# Autodesk Inventor assembly: ftc robot
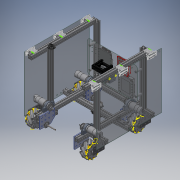
[picture p0: Inventor's stored thumbnail of the model, 180x180]
Saved by Autodesk Inventor 2017 (Build 210142000, 142)
## iProperties
Created: 2017-06-13
Part Number: ftc robot
Document SubType Name: Assembly
Designer: slong
Author: slong
## Documents named in this file (25)
- C:\Users\sfreisem-kirov\Documents\GitHub\ftc_app\Parts\ftc robot\ftc robot.iam
- C:\Users\sfreisem-kirov\Documents\GitHub\ftc_app\Parts\ftc robot\10HoleExtrudedPlate.STL.ipt
- C:\Users\sfreisem-kirov\Documents\GitHub\ftc_app\Parts\ftc robot\100mm Aluminum Mecanum wheels.ipt
- C:\Users\sfreisem-kirov\Documents\GitHub\ftc_app\Parts\ftc robot\extruded aluminum (4in).ipt
- C:\Users\sfreisem-kirov\Documents\GitHub\ftc_app\Parts\ftc robot\extruded aluminum (vertical).ipt
- C:\Users\sfreisem-kirov\Documents\GitHub\ftc_app\Parts\ftc robot\extruded aluminum (horizontal).ipt
- C:\Users\sfreisem-kirov\Documents\GitHub\ftc_app\Parts\ftc robot\8020 L bracket.ipt
- C:\Users\sfreisem-kirov\Documents\GitHub\ftc_app\Parts\ftc robot\Motor Bracket.ipt
- C:\Users\sfreisem-kirov\Documents\GitHub\ftc_app\Parts\ftc robot\Andymark Motor.ipt
- C:\Users\sfreisem-kirov\Documents\GitHub\ftc_app\Parts\ftc robot\8020 small L bracket.ipt
- C:\Users\sfreisem-kirov\Documents\GitHub\ftc_app\Parts\ftc robot\extracted\tetrix_739079_2012.iam
- C:\Users\sfreisem-kirov\Documents\GitHub\ftc_app\Parts\ftc robot\175mm 6mm D axle.ipt
- C:\Users\sfreisem-kirov\Documents\GitHub\ftc_app\Parts\ftc robot\extracted\tetrix_739165_2012.ipt
- C:\Users\sfreisem-kirov\Documents\GitHub\ftc_app\Parts\ftc robot\circuit board correct.ipt
- C:\Users\sfreisem-kirov\Documents\GitHub\ftc_app\Parts\ftc robot\MRI45-2200_Power_Distribution_Module.ipt
- C:\Users\sfreisem-kirov\Documents\GitHub\ftc_app\Parts\ftc robot\MRI45-2203_Motor_Controller.ipt
- C:\Users\sfreisem-kirov\Documents\GitHub\ftc_app\Parts\ftc robot\MRI45-2204_Servo_Controller.ipt
- C:\Users\sfreisem-kirov\Documents\GitHub\ftc_app\Parts\ftc robot\spacer2.ipt
- C:\Users\sfreisem-kirov\Documents\GitHub\ftc_app\Parts\ftc robot\45-2003_Compass.ipt
- C:\Users\sfreisem-kirov\Documents\GitHub\ftc_app\Parts\ftc robot\45-2018_Color.ipt
- C:\Users\sfreisem-kirov\Documents\GitHub\ftc_app\Parts\ftc robot\extracted\tetrix_739070_2012.ipt
- C:\Users\sfreisem-kirov\Documents\GitHub\ftc_app\Parts\ftc robot\side shield.ipt
- C:\Users\sfreisem-kirov\Documents\GitHub\ftc_app\Parts\ftc robot\45-2017_IRSeekerV3.ipt
- C:\Users\sfreisem-kirov\Documents\GitHub\ftc_app\Parts\ftc robot\ShieldSlideAttachment2-SFK.ipt
- C:\Users\sfreisem-kirov\Documents\GitHub\ftc_app\Parts\phoneHolder\PhoneFlipper1-SFK.iam
## Components (81 placed, 24 different names)
1. 10HoleExtrudedPlate.STL:1 — Mate:7, Mate:8, Flush:10, Mate:33, Mate:65
2. 10HoleExtrudedPlate.STL:2 — Mate:9, Mate:10, Flush:10, Flush:16, Mate:20, Mate:70
3. 10HoleExtrudedPlate.STL:3 — Mate:14, Flush:15, Mate:16, Flush:18, Mate:56, Mate:64
4. 10HoleExtrudedPlate.STL:4 — Mate:13, Flush:14, Flush:16, Flush:18, Mate:18, Mate:19, Mate:68
5. 100mm Aluminum Mecanum wheels:1 — Mate:20, Mate:29, Mate:30, Rotation:7
6. 100mm Aluminum Mecanum wheels:2 — Mate:22, Mate:25, Mate:26, Rotation:2
7. 100mm Aluminum Mecanum wheels:3 — Mate:19, Mate:27, Mate:28, Rotation:8
8. 100mm Aluminum Mecanum wheels:4 — Mate:23, Mate:24, Rotation:6
9. extruded aluminum (4in):1 — Flush:11, Mate:11, Flush:13, Mate:17, Flush:19, Mate:50, Flush:35, Flush:66
10. extruded aluminum (4in):2 — Mate:12, Flush:12, Flush:13, Mate:15, Flush:17, Mate:48, Flush:34
11. extruded aluminum (vertical):1 — Mate:50, Mate:51, Flush:35
12. extruded aluminum (vertical):2 — Mate:48, Mate:49, Flush:34, Mate:122, Flush:69, Flush:70
13. extruded aluminum (vertical):3 — Mate:46, Flush:33, Mate:97, Mate:112
14. extruded aluminum (vertical):4 — Mate:44, Mate:45, Flush:32, Flush:46, Mate:98, Mate:111
15. extruded aluminum (horizontal):1 — Mate:2, Flush:2, Flush:3, Mate:3, Mate:8, Mate:12, Flush:12, Mate:14, Flush:15, Mate:36, Mate:37, Flush:23, Flush:24, Mate:44, Mate:49, Mate:53, Flush:58, Mate:119
16. extruded aluminum (horizontal):2 — Mate:1, Flush:1, Mate:2, Flush:2, Flush:4, Flush:5, Mate:4, Flush:6, Flush:7, Mate:5, Flush:8, Flush:9, Mate:45, Flush:32, Mate:46, Mate:113
17. extruded aluminum (horizontal):3 — Mate:1, Flush:1, Flush:3, Flush:4, Mate:9, Flush:11, Mate:11, Mate:13, Flush:14, Flush:22, Mate:34, Mate:35, Flush:25, Flush:33, Mate:51, Mate:54, Mate:97, Flush:57, Mate:117
18. extruded aluminum (horizontal):4 — Mate:3, Flush:5, Mate:52, Flush:36, Flush:37, Mate:55, Mate:113, Mate:114, Flush:59, Flush:62, Mate:118, Flush:63, Mate:120, Mate:121
19. 8020 L bracket:1 — Mate:5, Flush:8, Flush:9, Mate:10, Flush:30, Mate:58, Flush:41
20. 8020 L bracket:2 — Mate:15, Flush:17, Mate:16, Mate:22, Mate:31, Flush:29, Flush:38
21. 8020 L bracket:3 — Mate:4, Flush:6, Flush:7, Mate:7, Flush:28, Mate:59, Flush:39
22. 8020 L bracket:4 — Mate:17, Flush:19, Mate:18, Mate:32, Flush:31, Mate:57, Flush:40
23. Motor Bracket:1 — Mate:36, Flush:24, Flush:26, Mate:40
24. Motor Bracket:2 — Mate:37, Flush:23, Flush:27, Mate:41
25. Motor Bracket:3 — Mate:35, Flush:25, Flush:26, Mate:39
26. Motor Bracket:4 — Flush:22, Mate:34, Flush:27, Mate:38
27. Andymark Motor:1 — Mate:38, Mate:43, Flush:30, Mate:72, Mate:94
28. Andymark Motor:2 — Mate:39, Mate:42, Flush:31, Mate:69, Mate:76
29. Andymark Motor:3 — Mate:40, Mate:42, Flush:29, Mate:63, Mate:82
30. Andymark Motor:4 — Mate:41, Mate:43, Flush:28, Mate:67, Mate:88
31. 8020 small L bracket:1 — Mate:54, Flush:37, Mate:55
32. 8020 small L bracket:4 — Mate:52, Flush:36, Mate:53
33. tetrix_739079_2012:1 [sub-assembly] — Mate:25, Mate:26, Flush:21, Mate:31
34. tetrix_739079_2012:2 [sub-assembly] — Mate:23, Mate:24, Flush:21, Mate:33
35. tetrix_739079_2012:3 [sub-assembly] — Mate:27, Mate:28, Flush:20, Mate:32
36. tetrix_739079_2012:4 [sub-assembly] — Mate:29, Mate:30, Flush:20
37. tetrix_739079_2012:5 [sub-assembly] — Mate:60, Flush:42, Rotation:1, Rotation:2, Mate:64, Mate:80, Mate:81
38. tetrix_739079_2012:6 [sub-assembly] — Mate:69, Flush:44, Rotation:4, Mate:77, Mate:78
39. tetrix_739079_2012:7 [sub-assembly] — Mate:61, Mate:68, Flush:44, Rotation:4, Rotation:8, Mate:73, Mate:74, Mate:75
40. tetrix_739079_2012:9 [sub-assembly] — Mate:65, Mate:66, Flush:43, Rotation:5, Rotation:6, Mate:86, Mate:87
41. tetrix_739079_2012:10 [sub-assembly] — Mate:67, Flush:43, Rotation:5, Mate:89, Mate:90
42. tetrix_739079_2012:11 [sub-assembly] — Mate:70, Mate:71, Flush:45, Rotation:3, Rotation:7, Mate:92, Mate:93
43. tetrix_739079_2012:12 [sub-assembly] — Mate:72, Flush:45, Rotation:3, Mate:95, Mate:96
44. tetrix_739079_2012:8 [sub-assembly] — Mate:63, Flush:42, Rotation:1, Mate:83, Mate:84
45. 175mm 6mm D axle:1 — Mate:56, Flush:38, Mate:60, Mate:79
46. 175mm 6mm D axle:2 — Mate:57, Flush:40, Mate:61
47. 175mm 6mm D axle:3 — Mate:59, Flush:39, Mate:66, Mate:85
48. 175mm 6mm D axle:4 — Mate:58, Flush:41, Mate:71, Mate:91
49. tetrix_739165_2012:1 — Mate:76, Mate:77, Mate:78
50. tetrix_739165_2012:2 — Mate:85, Mate:86, Mate:87
51. tetrix_739165_2012:3 — Mate:91, Mate:92, Mate:93
52. tetrix_739165_2012:4 — Mate:82, Mate:83, Mate:84
53. tetrix_739165_2012:5 — Mate:79, Mate:80, Mate:81
54. tetrix_739165_2012:6 — Mate:88, Mate:89, Mate:90
55. tetrix_739165_2012:7 — Mate:94, Mate:95, Mate:96
56. tetrix_739165_2012:8 — Mate:73, Mate:74, Mate:75
57. circuit board correct:1 — Flush:46, Mate:98, Mate:99, Flush:47, Flush:48, Mate:100, Mate:101, Mate:102, Flush:49, Flush:50, Flush:51, Flush:52, Flush:53, Flush:54, Mate:103, Mate:104, Mate:105, Mate:106, Mate:107, Mate:108, Mate:109, Mate:110
58. MRI45-2200_Power_Distribution_Module:1 — Mate:99, Flush:47, Flush:48
59. MRI45-2203_Motor_Controller:1 — Mate:100, Flush:49, Flush:50
60. MRI45-2203_Motor_Controller:2 — Mate:101, Flush:53, Flush:54
61. MRI45-2204_Servo_Controller:1 — Mate:102, Flush:51, Flush:52
62. spacer2:1 — Mate:106, Mate:108
63. spacer2:2 — Mate:105, Mate:107
64. spacer2:3 — Mate:103, Mate:109
65. spacer2:4 — Mate:104, Mate:110
66. extruded aluminum (horizontal):7 — Mate:111, Flush:55, Flush:58, Flush:67, Flush:68, Mate:132, Mate:133, Mate:134
67. extruded aluminum (horizontal):8 — Mate:112, Flush:55, Flush:57, Flush:65, Mate:126, Mate:135, Mate:136, Mate:137, Mate:138
68. 45-2003_Compass:1 — Mate:117, Mate:118, Flush:63
69. 45-2018_Color:1 — Mate:115, Flush:60, Flush:61, Mate:116, Mate:119
70. 45-2018_Color:2 — Mate:115, Flush:60, Flush:61, Flush:62
71. tetrix_739070_2012:1 — Mate:114, Flush:59, Mate:116
72. side shield:2 — Mate:120, Flush:65, Flush:66, Mate:125, Mate:127, Mate:128
73. side shield:3 — Mate:121, Flush:67, Flush:68, Mate:129, Mate:130, Mate:131
74. 45-2017_IRSeekerV3:1 — Mate:122, Flush:69, Flush:70
75. ShieldSlideAttachment2-SFK:1 — Mate:125, Mate:126
76. ShieldSlideAttachment2-SFK:2 — Mate:128, Mate:136
77. ShieldSlideAttachment2-SFK:3 — Mate:129, Mate:132
78. ShieldSlideAttachment2-SFK:4 — Mate:127, Mate:135
79. ShieldSlideAttachment2-SFK:5 — Mate:131, Mate:133
80. ShieldSlideAttachment2-SFK:6 — Mate:130, Mate:134
81. PhoneFlipper1-SFK:1 [sub-assembly] — Mate:137, Mate:138
## Relationships (208: Mate 132, Flush 68, RelateRotation 8)
- Mate:1: extruded aluminum (horizontal):2 ↔ extruded aluminum (horizontal):3
- Flush:1 (-76.2 mm): extruded aluminum (horizontal):2 ↔ extruded aluminum (horizontal):3
- Mate:2: extruded aluminum (horizontal):1 ↔ extruded aluminum (horizontal):2
- Flush:2 (-76.2 mm): extruded aluminum (horizontal):1 ↔ extruded aluminum (horizontal):2
- Flush:3: extruded aluminum (horizontal):1 ↔ extruded aluminum (horizontal):3
- Flush:4: extruded aluminum (horizontal):2 ↔ extruded aluminum (horizontal):3
- Mate:3: extruded aluminum (horizontal):1 ↔ extruded aluminum (horizontal):4
- Flush:5: extruded aluminum (horizontal):2 ↔ extruded aluminum (horizontal):4
- Mate:4: extruded aluminum (horizontal):2 ↔ 8020 L bracket:3
- Flush:6: extruded aluminum (horizontal):2 ↔ 8020 L bracket:3
- Flush:7: extruded aluminum (horizontal):2 ↔ 8020 L bracket:3
- Mate:5: extruded aluminum (horizontal):2 ↔ 8020 L bracket:1
- Flush:8: extruded aluminum (horizontal):2 ↔ 8020 L bracket:1
- Flush:9: extruded aluminum (horizontal):2 ↔ 8020 L bracket:1
- Mate:7: 10HoleExtrudedPlate.STL:1 ↔ 8020 L bracket:3
- Mate:8: 10HoleExtrudedPlate.STL:1 ↔ extruded aluminum (horizontal):1
- Mate:9: 10HoleExtrudedPlate.STL:2 ↔ extruded aluminum (horizontal):3
- Mate:10: 10HoleExtrudedPlate.STL:2 ↔ 8020 L bracket:1
- Flush:10: 10HoleExtrudedPlate.STL:1 ↔ 10HoleExtrudedPlate.STL:2
- Flush:11: extruded aluminum (4in):1 ↔ extruded aluminum (horizontal):3
- Mate:11: extruded aluminum (4in):1 ↔ extruded aluminum (horizontal):3
- Mate:12: extruded aluminum (4in):2 ↔ extruded aluminum (horizontal):1
- Flush:12: extruded aluminum (4in):2 ↔ extruded aluminum (horizontal):1
- Flush:13: extruded aluminum (4in):1 ↔ extruded aluminum (4in):2
- Mate:13: 10HoleExtrudedPlate.STL:4 ↔ extruded aluminum (horizontal):3
- Flush:14: 10HoleExtrudedPlate.STL:4 ↔ extruded aluminum (horizontal):3
- Mate:14: 10HoleExtrudedPlate.STL:3 ↔ extruded aluminum (horizontal):1
- Flush:15: 10HoleExtrudedPlate.STL:3 ↔ extruded aluminum (horizontal):1
- Flush:16: 10HoleExtrudedPlate.STL:2 ↔ 10HoleExtrudedPlate.STL:4
- Mate:15: extruded aluminum (4in):2 ↔ 8020 L bracket:2
- Flush:17: extruded aluminum (4in):2 ↔ 8020 L bracket:2
- Mate:16: 10HoleExtrudedPlate.STL:3 ↔ 8020 L bracket:2
- Flush:18: 10HoleExtrudedPlate.STL:3 ↔ 10HoleExtrudedPlate.STL:4
- Mate:17: extruded aluminum (4in):1 ↔ 8020 L bracket:4
- Flush:19: extruded aluminum (4in):1 ↔ 8020 L bracket:4
- Mate:18: 10HoleExtrudedPlate.STL:4 ↔ 8020 L bracket:4
- Mate:19: 10HoleExtrudedPlate.STL:4 ↔ 100mm Aluminum Mecanum wheels:3
- Mate:20: 10HoleExtrudedPlate.STL:2 ↔ 100mm Aluminum Mecanum wheels:1
- Mate:22: 100mm Aluminum Mecanum wheels:2 ↔ 8020 L bracket:2
- Mate:23: 100mm Aluminum Mecanum wheels:4 ↔ tetrix_739079_2012:2
- Mate:24: 100mm Aluminum Mecanum wheels:4 ↔ tetrix_739079_2012:2
- Mate:25: 100mm Aluminum Mecanum wheels:2 ↔ tetrix_739079_2012:1
- Mate:26: 100mm Aluminum Mecanum wheels:2 ↔ tetrix_739079_2012:1
- Mate:27: 100mm Aluminum Mecanum wheels:3 ↔ tetrix_739079_2012:3
- Mate:28: 100mm Aluminum Mecanum wheels:3 ↔ tetrix_739079_2012:3
- Mate:29: 100mm Aluminum Mecanum wheels:1 ↔ tetrix_739079_2012:4
- Mate:30: 100mm Aluminum Mecanum wheels:1 ↔ tetrix_739079_2012:4
- Flush:20: tetrix_739079_2012:3 ↔ tetrix_739079_2012:4
- Flush:21: tetrix_739079_2012:1 ↔ tetrix_739079_2012:2
- Mate:31: 8020 L bracket:2 ↔ tetrix_739079_2012:1
- Mate:32: 8020 L bracket:4 ↔ tetrix_739079_2012:3
- Mate:33: 10HoleExtrudedPlate.STL:1 ↔ tetrix_739079_2012:2
- Flush:22 (6.35 mm): extruded aluminum (horizontal):3 ↔ Motor Bracket:4
- Mate:34: extruded aluminum (horizontal):3 ↔ Motor Bracket:4
- Mate:35: extruded aluminum (horizontal):3 ↔ Motor Bracket:3
- Mate:36: extruded aluminum (horizontal):1 ↔ Motor Bracket:1
- Mate:37: extruded aluminum (horizontal):1 ↔ Motor Bracket:2
- Flush:23 (6.35 mm): extruded aluminum (horizontal):1 ↔ Motor Bracket:2
- Flush:24 (6.35 mm): extruded aluminum (horizontal):1 ↔ Motor Bracket:1
- Flush:25 (6.35 mm): extruded aluminum (horizontal):3 ↔ Motor Bracket:3
- Flush:26: Motor Bracket:1 ↔ Motor Bracket:3
- Flush:27: Motor Bracket:2 ↔ Motor Bracket:4
- Mate:38: Motor Bracket:4 ↔ Andymark Motor:1
- Mate:39: Motor Bracket:3 ↔ Andymark Motor:2
- Mate:40: Motor Bracket:1 ↔ Andymark Motor:3
- Mate:41: Motor Bracket:2 ↔ Andymark Motor:4
- Mate:42: Andymark Motor:2 ↔ Andymark Motor:3
- Mate:43: Andymark Motor:1 ↔ Andymark Motor:4
- Flush:28: 8020 L bracket:3 ↔ Andymark Motor:4
- Flush:29: 8020 L bracket:2 ↔ Andymark Motor:3
- Flush:30: 8020 L bracket:1 ↔ Andymark Motor:1
- Flush:31: 8020 L bracket:4 ↔ Andymark Motor:2
- Mate:44: extruded aluminum (vertical):4 ↔ extruded aluminum (horizontal):1
- Mate:45: extruded aluminum (vertical):4 ↔ extruded aluminum (horizontal):2
- Flush:32: extruded aluminum (vertical):4 ↔ extruded aluminum (horizontal):2
- Mate:46: extruded aluminum (vertical):3 ↔ extruded aluminum (horizontal):2
- Flush:33: extruded aluminum (vertical):3 ↔ extruded aluminum (horizontal):3
- Mate:48: extruded aluminum (4in):2 ↔ extruded aluminum (vertical):2
- Mate:49: extruded aluminum (vertical):2 ↔ extruded aluminum (horizontal):1
- Flush:34: extruded aluminum (4in):2 ↔ extruded aluminum (vertical):2
- Mate:50: extruded aluminum (4in):1 ↔ extruded aluminum (vertical):1
- Mate:51: extruded aluminum (vertical):1 ↔ extruded aluminum (horizontal):3
- Flush:35: extruded aluminum (4in):1 ↔ extruded aluminum (vertical):1
- Mate:52: extruded aluminum (horizontal):4 ↔ 8020 small L bracket:4
- Flush:36 (1.5875 mm): extruded aluminum (horizontal):4 ↔ 8020 small L bracket:4
- Mate:53: extruded aluminum (horizontal):1 ↔ 8020 small L bracket:4
- Mate:54: extruded aluminum (horizontal):3 ↔ 8020 small L bracket:1
- Flush:37: extruded aluminum (horizontal):4 ↔ 8020 small L bracket:1
- Mate:55: extruded aluminum (horizontal):4 ↔ 8020 small L bracket:1
- Mate:56: 10HoleExtrudedPlate.STL:3 ↔ 175mm 6mm D axle:1
- Mate:57: 8020 L bracket:4 ↔ 175mm 6mm D axle:2
- Mate:58: 8020 L bracket:1 ↔ 175mm 6mm D axle:4
- Mate:59: 8020 L bracket:3 ↔ 175mm 6mm D axle:3
- Flush:38: 8020 L bracket:2 ↔ 175mm 6mm D axle:1
- Flush:39: 8020 L bracket:3 ↔ 175mm 6mm D axle:3
- Flush:40: 8020 L bracket:4 ↔ 175mm 6mm D axle:2
- Flush:41: 8020 L bracket:1 ↔ 175mm 6mm D axle:4
- Mate:60: tetrix_739079_2012:5 ↔ 175mm 6mm D axle:1
- Mate:61: tetrix_739079_2012:7 ↔ 175mm 6mm D axle:2
- Mate:63: Andymark Motor:3 ↔ tetrix_739079_2012:8
- Flush:42: tetrix_739079_2012:5 ↔ tetrix_739079_2012:8
- Rotation:1 [RelateRotation] (1 ul): tetrix_739079_2012:5 ↔ tetrix_739079_2012:8
- Rotation:2 [RelateRotation] (-1 ul): 100mm Aluminum Mecanum wheels:2 ↔ tetrix_739079_2012:5
- Mate:64: 10HoleExtrudedPlate.STL:3 ↔ tetrix_739079_2012:5
- Mate:65: 10HoleExtrudedPlate.STL:1 ↔ tetrix_739079_2012:9
- Mate:66: tetrix_739079_2012:9 ↔ 175mm 6mm D axle:3
- Mate:67: Andymark Motor:4 ↔ tetrix_739079_2012:10
- Flush:43: tetrix_739079_2012:9 ↔ tetrix_739079_2012:10
- Mate:68: 10HoleExtrudedPlate.STL:4 ↔ tetrix_739079_2012:7
- Mate:69: Andymark Motor:2 ↔ tetrix_739079_2012:6
- Flush:44: tetrix_739079_2012:6 ↔ tetrix_739079_2012:7
- Mate:70: 10HoleExtrudedPlate.STL:2 ↔ tetrix_739079_2012:11
- Mate:71: tetrix_739079_2012:11 ↔ 175mm 6mm D axle:4
- Mate:72: Andymark Motor:1 ↔ tetrix_739079_2012:12
- Flush:45: tetrix_739079_2012:11 ↔ tetrix_739079_2012:12
- Rotation:3 [RelateRotation] (1 ul): tetrix_739079_2012:11 ↔ tetrix_739079_2012:12
- Rotation:4 [RelateRotation] (1 ul): tetrix_739079_2012:6 ↔ tetrix_739079_2012:7
- Rotation:5 [RelateRotation] (1 ul): tetrix_739079_2012:9 ↔ tetrix_739079_2012:10
- Rotation:6 [RelateRotation] (-1 ul): 100mm Aluminum Mecanum wheels:4 ↔ tetrix_739079_2012:9
- Rotation:7 [RelateRotation] (-1 ul): 100mm Aluminum Mecanum wheels:1 ↔ tetrix_739079_2012:11
- Rotation:8 [RelateRotation] (-1 ul): 100mm Aluminum Mecanum wheels:3 ↔ tetrix_739079_2012:7
- Mate:73: tetrix_739079_2012:7 ↔ tetrix_739165_2012:8
- Mate:74: tetrix_739079_2012:7 ↔ tetrix_739165_2012:8
- Mate:75: tetrix_739079_2012:7 ↔ tetrix_739165_2012:8
- Mate:76: Andymark Motor:2 ↔ tetrix_739165_2012:1
- Mate:77: tetrix_739079_2012:6 ↔ tetrix_739165_2012:1
- Mate:78: tetrix_739079_2012:6 ↔ tetrix_739165_2012:1
- Mate:79: 175mm 6mm D axle:1 ↔ tetrix_739165_2012:5
- Mate:80: tetrix_739079_2012:5 ↔ tetrix_739165_2012:5
- Mate:81: tetrix_739079_2012:5 ↔ tetrix_739165_2012:5
- Mate:82: Andymark Motor:3 ↔ tetrix_739165_2012:4
- Mate:83: tetrix_739079_2012:8 ↔ tetrix_739165_2012:4
- Mate:84: tetrix_739079_2012:8 ↔ tetrix_739165_2012:4
- Mate:85: 175mm 6mm D axle:3 ↔ tetrix_739165_2012:2
- Mate:86: tetrix_739079_2012:9 ↔ tetrix_739165_2012:2
- Mate:87: tetrix_739079_2012:9 ↔ tetrix_739165_2012:2
- Mate:88: Andymark Motor:4 ↔ tetrix_739165_2012:6
- Mate:89: tetrix_739079_2012:10 ↔ tetrix_739165_2012:6
- Mate:90: tetrix_739079_2012:10 ↔ tetrix_739165_2012:6
- Mate:91: 175mm 6mm D axle:4 ↔ tetrix_739165_2012:3
- Mate:92: tetrix_739079_2012:11 ↔ tetrix_739165_2012:3
- Mate:93: tetrix_739079_2012:11 ↔ tetrix_739165_2012:3
- Mate:94: Andymark Motor:1 ↔ tetrix_739165_2012:7
- Mate:95: tetrix_739079_2012:12 ↔ tetrix_739165_2012:7
- Mate:96: tetrix_739079_2012:12 ↔ tetrix_739165_2012:7
- Mate:97: extruded aluminum (vertical):3 ↔ extruded aluminum (horizontal):3
- Flush:46 (1.524 mm): extruded aluminum (vertical):4 ↔ circuit board correct:1
- Mate:98 (38.1 mm): extruded aluminum (vertical):4 ↔ circuit board correct:1
- Mate:99: circuit board correct:1 ↔ MRI45-2200_Power_Distribution_Module:1
- Flush:47 (34.163 mm): circuit board correct:1 ↔ MRI45-2200_Power_Distribution_Module:1
- Flush:48 (4.9022 mm): circuit board correct:1 ↔ MRI45-2200_Power_Distribution_Module:1
- Mate:100: circuit board correct:1 ↔ MRI45-2203_Motor_Controller:1
- Mate:101: circuit board correct:1 ↔ MRI45-2203_Motor_Controller:2
- Mate:102: circuit board correct:1 ↔ MRI45-2204_Servo_Controller:1
- Flush:49 (25.6794 mm): circuit board correct:1 ↔ MRI45-2203_Motor_Controller:1
- Flush:50 (180.9242 mm): circuit board correct:1 ↔ MRI45-2203_Motor_Controller:1
- Flush:51 (9.2202 mm): circuit board correct:1 ↔ MRI45-2204_Servo_Controller:1
- Flush:52 (200.4568 mm): circuit board correct:1 ↔ MRI45-2204_Servo_Controller:1
- Flush:53 (124.5362 mm): circuit board correct:1 ↔ MRI45-2203_Motor_Controller:2
- Flush:54 (51.7906 mm): circuit board correct:1 ↔ MRI45-2203_Motor_Controller:2
- Mate:103: circuit board correct:1 ↔ spacer2:3
- Mate:104: circuit board correct:1 ↔ spacer2:4
- Mate:105: circuit board correct:1 ↔ spacer2:2
- Mate:106: circuit board correct:1 ↔ spacer2:1
- Mate:107: circuit board correct:1 ↔ spacer2:2
- Mate:108: circuit board correct:1 ↔ spacer2:1
- Mate:109: circuit board correct:1 ↔ spacer2:3
- Mate:110: circuit board correct:1 ↔ spacer2:4
- Mate:111: extruded aluminum (vertical):4 ↔ extruded aluminum (horizontal):7
- Mate:112: extruded aluminum (vertical):3 ↔ extruded aluminum (horizontal):8
- Flush:55: extruded aluminum (horizontal):7 ↔ extruded aluminum (horizontal):8
- Flush:57: extruded aluminum (horizontal):3 ↔ extruded aluminum (horizontal):8
- Flush:58: extruded aluminum (horizontal):1 ↔ extruded aluminum (horizontal):7
- Mate:113 (-180.975 mm): extruded aluminum (horizontal):2 ↔ extruded aluminum (horizontal):4
- Mate:114: extruded aluminum (horizontal):4 ↔ tetrix_739070_2012:1
- Flush:59 (3.175 mm): extruded aluminum (horizontal):4 ↔ tetrix_739070_2012:1
- Mate:115: 45-2018_Color:1 ↔ 45-2018_Color:2
- Flush:60: 45-2018_Color:1 ↔ 45-2018_Color:2
- Flush:61: 45-2018_Color:1 ↔ 45-2018_Color:2
- Mate:116: 45-2018_Color:1 ↔ tetrix_739070_2012:1
- Flush:62 (-3.175 mm): extruded aluminum (horizontal):4 ↔ 45-2018_Color:2
- Mate:117 (104.775 mm): extruded aluminum (horizontal):3 ↔ 45-2003_Compass:1
- Mate:118: extruded aluminum (horizontal):4 ↔ 45-2003_Compass:1
- Flush:63 (9.525 mm): extruded aluminum (horizontal):4 ↔ 45-2003_Compass:1
- Mate:119 (88.9 mm): extruded aluminum (horizontal):1 ↔ 45-2018_Color:1
- Mate:120: extruded aluminum (horizontal):4 ↔ side shield:2
- Flush:65: extruded aluminum (horizontal):8 ↔ side shield:2
- Flush:66: extruded aluminum (4in):1 ↔ side shield:2
- Mate:121: extruded aluminum (horizontal):4 ↔ side shield:3
- Flush:67: extruded aluminum (horizontal):7 ↔ side shield:3
- Flush:68: extruded aluminum (horizontal):7 ↔ side shield:3
- Mate:122: extruded aluminum (vertical):2 ↔ 45-2017_IRSeekerV3:1
- Flush:69: extruded aluminum (vertical):2 ↔ 45-2017_IRSeekerV3:1
- Flush:70: extruded aluminum (vertical):2 ↔ 45-2017_IRSeekerV3:1
- Mate:125: side shield:2 ↔ ShieldSlideAttachment2-SFK:1
- Mate:126: extruded aluminum (horizontal):8 ↔ ShieldSlideAttachment2-SFK:1
- Mate:127: side shield:2 ↔ ShieldSlideAttachment2-SFK:4
- Mate:128: side shield:2 ↔ ShieldSlideAttachment2-SFK:2
- Mate:129: side shield:3 ↔ ShieldSlideAttachment2-SFK:3
- Mate:130: side shield:3 ↔ ShieldSlideAttachment2-SFK:6
- Mate:131: side shield:3 ↔ ShieldSlideAttachment2-SFK:5
- Mate:132: extruded aluminum (horizontal):7 ↔ ShieldSlideAttachment2-SFK:3
- Mate:133: extruded aluminum (horizontal):7 ↔ ShieldSlideAttachment2-SFK:5
- Mate:134: extruded aluminum (horizontal):7 ↔ ShieldSlideAttachment2-SFK:6
- Mate:135: extruded aluminum (horizontal):8 ↔ ShieldSlideAttachment2-SFK:4
- Mate:136: extruded aluminum (horizontal):8 ↔ ShieldSlideAttachment2-SFK:2
- Mate:137: extruded aluminum (horizontal):8 ↔ PhoneFlipper1-SFK:1
- Mate:138: extruded aluminum (horizontal):8 ↔ PhoneFlipper1-SFK:1
